# Autodesk Inventor assembly: Guida a terra
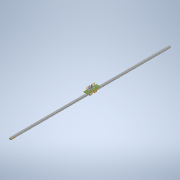
[picture p0: Inventor's stored thumbnail of the model, 180x180]
Saved by Autodesk Inventor 2022 (Build 260153000, 153)
## iProperties
RuleStatus: InUse
Part Number: Guida a terra
Document SubType Name: Assieme
Designer: matte
Author: matte
## Documents named in this file (5)
- C:\Users\matte\Documents\GitHub\MDM-CyberOrto-CAD\Guida a terra.iam
- C:\Users\matte\Documents\GitHub\MDM-CyberOrto-CAD\Pezzi singoli\Supporto lineare\Binario.ipt
- C:\Users\matte\Documents\GitHub\MDM-CyberOrto-CAD\Pezzi singoli\Supporto lineare\Clamp.ipt
- C:\Users\matte\Documents\GitHub\MDM-CyberOrto-CAD\Pezzi singoli\Supporto lineare\Shaft.ipt
- C:\Users\matte\Documents\GitHub\MDM-CyberOrto-CAD\Pezzi singoli\Supporto lineare\Guida con supporto.iam
## Components (6 placed, 6 different names)
1. Binario:1 — Coincidente:1, Coincidente:2, Coincidente:3, Allineato:1, Coincidente:4, Coincidente:5, Coincidente:7, Coincidente:8
2. Clamp DX — Allineato:1, Coincidente:4, Coincidente:5, Allineato:2, Allineato:3, Tangente:1, Simmetria:1
3. Shaft DX — Allineato:2, Allineato:3, Tangente:1, Allineato:6, Allineato:7
4. Clamp SX — Simmetria:1
5. Shaft SX — Allineato:6, Allineato:7
6. Guida con supporto:1 [sub-assembly] — Coincidente:7, Coincidente:8
## Relationships (17: Mate 7, Flush 7, Tangent 2, Symmetry 1)
- Coincidente:1 [Mate]: Binario:1
- Coincidente:2 [Mate]: Binario:1
- Coincidente:3 [Mate]: Binario:1
- Allineato:1 [Flush]: Binario:1 ↔ Clamp DX
- Coincidente:4 [Mate]: Binario:1 ↔ Clamp DX
- Coincidente:5 [Mate]: Binario:1 ↔ Clamp DX
- Allineato:2 [Flush]: Clamp DX ↔ Shaft DX
- Allineato:3 [Flush]: Clamp DX ↔ Shaft DX
- Tangente:1: Clamp DX ↔ Shaft DX
- [Flush]: Clamp SX ↔ Shaft SX
- [Flush]: Clamp SX ↔ Shaft SX
- [Tangent]: Clamp SX ↔ Shaft SX
- Simmetria:1 [Symmetry]: Clamp DX ↔ Clamp SX
- Allineato:6 [Flush]: Shaft DX ↔ Shaft SX
- Allineato:7 [Flush]: Shaft DX ↔ Shaft SX
- Coincidente:7 [Mate] (20 mm): Binario:1 ↔ Guida con supporto:1
- Coincidente:8 [Mate] (-40 mm): Binario:1 ↔ Guida con supporto:1
## Named parameters: L_traccia = 4000 mm, d11_d8 = 0 mm, d12_d9 = 0 mm, d13_d10 = 0 mm, L_piatto = 240 mm
